# Autodesk Inventor assembly: PasekZKolamiNowy
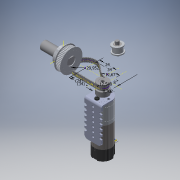
[picture p0: Inventor's stored thumbnail of the model, 180x180]
Saved by Autodesk Inventor 2019 (Build 230136000, 136)
## iProperties
Created: 2020-08-21
Part Number: PasekZKolamiNowy
Document SubType Name: Assembly
Designer: estee
Author: estee
## Documents named in this file (5)
- C:\Users\estee\OneDrive\Pulpit\estere\1\MUM\projejt\PasekZKolamiNowy.iam
- C:\Users\estee\OneDrive\Pulpit\estere\1\MUM\projejt\PasekZebatyNowy.iam
- C:\Users\estee\OneDrive\Pulpit\estere\1\MUM\projejt\ModulDuzegoKola.iam
- C:\Users\estee\OneDrive\Pulpit\estere\1\MUM\projejt\ModulSilnika.iam
- C:\Users\estee\OneDrive\Pulpit\estere\1\MUM\projejt\ModulKolaNapinajacego.iam
## Components (4 placed, 4 different names)
1. PasekZebatyNowy:1 [sub-assembly] — Mate:1, Mate:2
2. ModulDuzegoKola:1 [sub-assembly]
3. ModulSilnika:1 [sub-assembly] — Mate:1, Mate:2
4. ModulKolaNapinajacego:1 [sub-assembly]
## Relationships (2: Mate 2)
- Mate:1: PasekZebatyNowy:1 ↔ ModulSilnika:1
- Mate:2 (0.5 mm): PasekZebatyNowy:1 ↔ ModulSilnika:1
